# Autodesk Inventor assembly: OpticsTable_Shelf
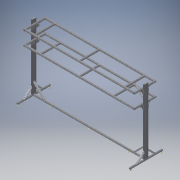
[picture p0: Inventor's stored thumbnail of the model, 180x180]
Saved by Autodesk Inventor 2018 (Build 220112000, 112)
## iProperties
Created: 2018-01-27
Part Number: OpticsTable_Shelf
Document SubType Name: Assembly
Designer: Rich
Author: Rich
## Documents named in this file (23)
- C:\Users\Rich\development\UWaterloo\opticstable_shelf\OpticsTable_Shelf.iam
- C:\Users\Rich\development\UWaterloo\opticstable_shelf\8020-1545-S-1545-S X 54.ipt
- C:\Users\Rich\development\UWaterloo\opticstable_shelf\8020-1515-LS-1515-LS X 24.ipt
- C:\Users\Rich\development\UWaterloo\opticstable_shelf\8020-1515-LS-1515-LS X 21.ipt
- C:\Users\Rich\development\UWaterloo\opticstable_shelf\8020 Original Parts\8020-3660-DEFAULT.ipt
- C:\Users\Rich\development\UWaterloo\opticstable_shelf\8020-1515-LS-1515-LS X 36.ipt
- C:\Users\Rich\development\UWaterloo\opticstable_shelf\8020 Original Parts\8020-2561-$PARTNUMBER.ipt
- C:\Users\Rich\development\UWaterloo\opticstable_shelf\8020 Original Parts\8020-2563-$PARTNUMBER.ipt
- C:\Users\Rich\development\UWaterloo\opticstable_shelf\8020 Original Parts\8020-2190-DEFAULT.ipt
- C:\Users\Rich\development\UWaterloo\opticstable_shelf\8020 Original Parts\8020-2200-DEFAULT.ipt
- C:\Users\Rich\development\UWaterloo\opticstable_shelf\8020 Original Parts\RS2000-410-12.ipt
- C:\Users\Rich\development\UWaterloo\opticstable_shelf\8020 Original Parts\Newport SL 1200-422.ipt
- C:\Users\Rich\development\UWaterloo\opticstable_shelf\8020-1515-LS-1515-LS X 120.ipt
- C:\Users\Rich\development\UWaterloo\opticstable_shelf\8020-1515-LS-1515-LS X 123.ipt
- C:\Users\Rich\development\UWaterloo\opticstable_shelf\8020 Original Parts\8020-3118-DEFAULT.ipt
- C:\Users\Rich\development\UWaterloo\opticstable_shelf\8020 Original Parts\8020-4461-DEFAULT.ipt
- C:\Users\Rich\development\UWaterloo\opticstable_shelf\8020 Original Parts\8020-4336-BLACK-DEFAULT.ipt
- C:\Users\Rich\development\UWaterloo\opticstable_shelf\8020 Original Parts\User Library-ANSI - BHCS - 0.625_5.5.ipt
- C:\Users\Rich\development\UWaterloo\opticstable_shelf\8020 Original Parts\8020-3202-DEFAULT.ipt
- C:\Users\Rich\development\UWaterloo\opticstable_shelf\8020 Original Parts\8020-3065-DEFAULT.ipt
- C:\Users\Rich\development\UWaterloo\opticstable_shelf\8020 Original Parts\8020-2046-DEFAULT.ipt
- C:\Users\Rich\development\UWaterloo\opticstable_shelf\8020 Original Parts\8020-2030-Plain-DEFAULT.ipt
- C:\Users\Rich\development\UWaterloo\opticstable_shelf\8020 Original Parts\8020-3214-DEFAULT.ipt
## Components (176 placed, 22 different names)
1. 8020-1545-S-1545-S X 54:1 — Mate:12, Flush:22, Flush:26, Mate:18, Mate:25, Flush:29, Mate:26, Flush:33, Flush:41, Mate:36, Angle:10, Flush:42, Mate:37, Angle:11, Mate:50, Flush:53, Mate:81, Mate:82, Mate:118, Mate:120, Mate:167, Mate:168, Mate:169, Mate:337, Mate:338, Mate:339, Mate:340
2. 8020-1545-S-1545-S X 54:2 — Mate:205, Flush:97, Mate:206, Mate:207, Mate:208, Flush:98, Mate:209, Mate:210, Mate:211, Tangent:5, Mate:212, Mate:213, Mate:285, Mate:286, Mate:287, Mate:288, Mate:341, Flush:126, Flush:127
3. 8020-1515-LS-1515-LS X 36:1 — Mate:12, Flush:19, Flush:22, Mate:24, Mate:27, Flush:30, Mate:38, Flush:43, Mate:39, Flush:44, Flush:77, Mate:75, Mate:175, Flush:85, Flush:86, Mate:176, Flush:87, Flush:88
4. 8020-1515-LS-1515-LS X 36:2 — Mate:1, Flush:19, Mate:20, Mate:22, Flush:28, Mate:40, Flush:45, Mate:41, Flush:46, Mate:72, Flush:75, Mate:173, Flush:81, Flush:82, Mate:174, Flush:83, Flush:84, Mate:205, Flush:97, Flush:98
5. 8020-2561-$PARTNUMBER:1 — Mate:22, Flush:28
6. 8020-2561-$PARTNUMBER:2 — Mate:24, Mate:25, Flush:29
7. 8020-2563-$PARTNUMBER:1 — Mate:17, Tangent:1, Mate:67, Mate:211, Tangent:5
8. 8020-2563-$PARTNUMBER:2 — Mate:18, Mate:19, Flush:33, Mate:68, Tangent:2
9. 8020-2561-$PARTNUMBER:3 — Mate:26, Mate:27, Flush:30
10. 8020-2561-$PARTNUMBER:4 — Mate:20
11. 8020-2190-DEFAULT:1
12. 8020-2190-DEFAULT:2
13. 8020-2190-DEFAULT:3
14. 8020-3660-DEFAULT:9
15. 8020-3660-DEFAULT:10
16. 8020-3660-DEFAULT:11 — Flush:41, Mate:36, Angle:10
17. 8020-3660-DEFAULT:12 — Flush:42, Mate:37, Angle:11
18. 8020-2200-DEFAULT:1 — Mate:38, Flush:43
19. 8020-2200-DEFAULT:2 — Mate:39, Flush:44
20. 8020-2200-DEFAULT:3 — Mate:40, Flush:45
21. 8020-2200-DEFAULT:4 — Mate:41, Flush:46
22. 8020-2563-$PARTNUMBER:3 — Flush:76, Mate:73
23. 8020-2563-$PARTNUMBER:4 — Mate:50, Flush:53, Mate:74
24. 8020-2200-DEFAULT:5 — Mate:76, Flush:78
25. 8020-2200-DEFAULT:6 — Flush:79, Mate:77
26. RS2000-410-12:1 — Mate:57, Mate:58, Flush:60
27. 8020-1515-LS-1515-LS X 123:1 — Mate:72, Flush:75, Flush:76, Mate:73, Mate:74, Flush:77, Mate:75, Mate:76, Flush:78, Flush:79, Mate:77, Mate:78, Flush:80
28. 8020-2200-DEFAULT:7 — Mate:78, Flush:80
29. 8020-2046-DEFAULT:1 — Mate:167, Mate:168, Mate:169
30. 8020-2046-DEFAULT:2 — Mate:206, Mate:207, Mate:208
31. 8020-2030-Plain-DEFAULT:5 — Mate:173, Flush:81, Flush:82
32. 8020-2030-Plain-DEFAULT:6 — Mate:174, Flush:83, Flush:84
33. 8020-2030-Plain-DEFAULT:7 — Mate:175, Flush:85, Flush:86
34. 8020-2030-Plain-DEFAULT:8 — Mate:176, Flush:87, Flush:88
35. 8020-1515-LS-1515-LS X 24:1 — Flush:61, Mate:60, Flush:62, Mate:61, Flush:63, Flush:64, Mate:129, Mate:179, Flush:93, Flush:94, Mate:180, Flush:95, Flush:96
36. 8020-1515-LS-1515-LS X 24:2 — Flush:23, Flush:68, Mate:64, Flush:69, Mate:130, Mate:177, Flush:89, Flush:90, Flush:91, Mate:178, Flush:92, Flush:127
37. 8020-1515-LS-1515-LS X 21:1 — Mate:17, Mate:46, Flush:51, Angle:16, Mate:47, Mate:48, Angle:17, Flush:72, Mate:68, Tangent:2, Mate:71
38. 8020-1515-LS-1515-LS X 21:2 — Flush:23, Mate:44, Flush:49, Angle:14, Mate:45, Flush:50, Angle:15, Flush:67, Mate:63
39. 8020-1515-LS-1515-LS X 21:3 — Mate:19, Flush:47, Mate:42, Angle:12, Flush:48, Mate:43, Angle:13, Mate:62, Flush:65, Tangent:1, Mate:67
40. 8020-3660-DEFAULT:1 — Mate:66, Flush:71, Angle:18
41. 8020-3660-DEFAULT:2 — Mate:69, Flush:73, Angle:19
42. 8020-3660-DEFAULT:3 — Mate:70, Flush:74, Angle:20
43. 8020-3660-DEFAULT:4 — Mate:65, Flush:70
44. 8020-3660-DEFAULT:13 — Flush:47, Mate:42, Angle:12
45. 8020-3660-DEFAULT:14 — Flush:48, Mate:43, Angle:13
46. 8020-3660-DEFAULT:15 — Mate:44, Flush:49, Angle:14
47. 8020-3660-DEFAULT:16 — Mate:45, Flush:50, Angle:15
48. 8020-3660-DEFAULT:17 — Mate:46, Flush:51, Angle:16
49. 8020-3660-DEFAULT:18 — Mate:47, Mate:48, Angle:17
50. 8020-1515-LS-1515-LS X 120:1 — Flush:62, Mate:61, Flush:63, Mate:63, Mate:66, Flush:71, Angle:18, Mate:69, Flush:73, Angle:19, Mate:71
51. 8020-1515-LS-1515-LS X 120:2 — Flush:61, Mate:60, Flush:64, Mate:62, Flush:65, Flush:67, Flush:68, Mate:64, Flush:69, Mate:65, Flush:70, Flush:72, Mate:70, Flush:74, Angle:20
52. 8020-2030-Plain-DEFAULT:1 — Mate:180, Flush:95, Flush:96
53. 8020-2030-Plain-DEFAULT:2 — Mate:179, Flush:93, Flush:94
54. 8020-2030-Plain-DEFAULT:3 — Flush:91, Mate:178, Flush:92
55. 8020-2030-Plain-DEFAULT:4 — Mate:177, Flush:89, Flush:90
56. 8020-3118-DEFAULT:1 — Mate:84, Mate:85, Mate:88, Mate:184
57. 8020-4461-DEFAULT:1 — Mate:95, Mate:96, Mate:97, Mate:116, Mate:117, Mate:123, Mate:124, Mate:193, Mate:194, Mate:213
58. 8020-4461-DEFAULT:2 — Mate:83, Mate:88, Mate:89, Mate:127, Mate:128, Mate:195, Mate:196, Mate:198, Mate:200, Mate:212
59. 8020-4336-BLACK-DEFAULT:1 — Mate:83, Mate:84, Mate:85, Mate:86, Mate:87, Mate:130, Mate:149, Mate:150, Mate:154, Mate:155, Mate:156
60. 8020-3118-DEFAULT:2 — Mate:86, Mate:87, Mate:89, Mate:185
61. 8020-4336-BLACK-DEFAULT:2 — Mate:91, Mate:92, Mate:93, Mate:94, Mate:95, Mate:151, Mate:152, Mate:153, Mate:157, Mate:158
62. 8020-3118-DEFAULT:3 — Mate:91, Mate:92, Mate:97, Mate:186
63. 8020-3118-DEFAULT:4 — Mate:93, Mate:94, Mate:96, Mate:187
64. User Library-ANSI - BHCS - 0.625_5.5:3 — Mate:117, Mate:124, Mate:128, Mate:199, Mate:210
65. User Library-ANSI - BHCS - 0.625_5.5:4 — Mate:116, Mate:123, Mate:127, Mate:197, Mate:209
66. 8020-3202-DEFAULT:6
67. 8020-3065-DEFAULT:6 — Mate:151, Mate:157, Mate:158
68. 8020-3202-DEFAULT:7
69. 8020-3065-DEFAULT:7 — Mate:150, Mate:155, Mate:156
70. 8020-3202-DEFAULT:8
71. 8020-3065-DEFAULT:8 — Mate:149, Mate:154
72. 8020-3202-DEFAULT:9
73. 8020-3065-DEFAULT:9 — Mate:152, Mate:153
74. 8020-3214-DEFAULT:4 — Mate:185, Mate:196
75. 8020-3214-DEFAULT:5 — Mate:184, Mate:195
76. 8020-3214-DEFAULT:6 — Mate:186, Mate:193
77. 8020-3214-DEFAULT:7 — Mate:187, Mate:194
78. 8020-3214-DEFAULT:9 — Mate:197, Mate:198
79. 8020-3214-DEFAULT:10 — Mate:199, Mate:200
80. 8020-4461-DEFAULT:3 — Mate:81, Mate:109, Mate:110, Mate:111, Mate:112, Mate:114, Mate:115, Mate:119, Mate:189, Mate:190
81. 8020-4461-DEFAULT:4 — Mate:82, Mate:102, Mate:103, Mate:104, Mate:121, Mate:122, Mate:191, Mate:192, Mate:202, Mate:204
82. 8020-3118-DEFAULT:5 — Mate:98, Mate:99, Mate:104, Mate:181
83. 8020-4336-BLACK-DEFAULT:3 — Mate:98, Mate:99, Mate:100, Mate:101, Mate:102, Mate:129, Mate:159, Mate:160, Mate:161, Mate:162
84. 8020-3118-DEFAULT:6 — Mate:100, Mate:101, Mate:103, Mate:182
85. 8020-4336-BLACK-DEFAULT:4 — Mate:105, Mate:106, Mate:107, Mate:108, Mate:109, Mate:163, Mate:164, Mate:165, Mate:166
86. 8020-3118-DEFAULT:7 — Mate:105, Mate:106, Mate:110, Mate:183
87. 8020-3118-DEFAULT:8 — Mate:107, Mate:108, Mate:111, Mate:188
88. User Library-ANSI - BHCS - 0.625_5.5:1 — Mate:114, Mate:115, Mate:118, Mate:121, Mate:203
89. User Library-ANSI - BHCS - 0.625_5.5:2 — Mate:112, Mate:119, Mate:120, Mate:122, Mate:201
90. 8020-3202-DEFAULT:1 — Mate:131, Mate:132
91. 8020-3065-DEFAULT:1 — Mate:131, Mate:132, Mate:159, Mate:160
92. 8020-3202-DEFAULT:2
93. 8020-3065-DEFAULT:2 — Mate:163, Mate:164
94. 8020-3202-DEFAULT:4
95. 8020-3065-DEFAULT:4 — Mate:165, Mate:166
96. 8020-3202-DEFAULT:5
97. 8020-3065-DEFAULT:5 — Mate:161, Mate:162
98. 8020-3214-DEFAULT:1 — Mate:181, Mate:191
99. 8020-3214-DEFAULT:2 — Mate:182, Mate:192
100. 8020-3214-DEFAULT:3 — Mate:183, Mate:190
101. 8020-3214-DEFAULT:8 — Mate:188, Mate:189
102. 8020-3214-DEFAULT:11 — Mate:201, Mate:202
103. 8020-3214-DEFAULT:12 — Mate:203, Mate:204
104. 8020-1515-LS-1515-LS X 24:3
105. 8020-1515-LS-1515-LS X 24:4 — Mate:341, Mate:342, Flush:126
106. 8020-1515-LS-1515-LS X 21:4
107. 8020-1515-LS-1515-LS X 21:5
108. 8020-1515-LS-1515-LS X 21:6
109. 8020-3660-DEFAULT:19
110. 8020-3660-DEFAULT:20
111. 8020-3660-DEFAULT:21
112. 8020-3660-DEFAULT:22
113. 8020-3660-DEFAULT:23
114. 8020-3660-DEFAULT:24
115. 8020-3660-DEFAULT:25
116. 8020-3660-DEFAULT:26
117. 8020-3660-DEFAULT:27
118. 8020-3660-DEFAULT:28
119. 8020-1515-LS-1515-LS X 120:3
120. 8020-1515-LS-1515-LS X 120:4
121. 8020-2030-Plain-DEFAULT:9
122. 8020-2030-Plain-DEFAULT:10
123. 8020-2030-Plain-DEFAULT:11
124. 8020-2030-Plain-DEFAULT:12
125. 8020-3118-DEFAULT:9
126. 8020-4461-DEFAULT:5 — Mate:286
127. 8020-4461-DEFAULT:6 — Mate:285
128. 8020-4336-BLACK-DEFAULT:5
129. 8020-3118-DEFAULT:10
130. 8020-4336-BLACK-DEFAULT:6 — Mate:342
131. 8020-3118-DEFAULT:11
132. 8020-3118-DEFAULT:12
133. User Library-ANSI - BHCS - 0.625_5.5:5 — Mate:287
134. User Library-ANSI - BHCS - 0.625_5.5:6 — Mate:288
135. 8020-3202-DEFAULT:10
136. 8020-3065-DEFAULT:10
137. 8020-3202-DEFAULT:11
138. 8020-3065-DEFAULT:11
139. 8020-3202-DEFAULT:12
140. 8020-3065-DEFAULT:12
141. 8020-3202-DEFAULT:13
142. 8020-3065-DEFAULT:13
143. 8020-3214-DEFAULT:13
144. 8020-3214-DEFAULT:14
145. 8020-3214-DEFAULT:15
146. 8020-3214-DEFAULT:16
147. 8020-3214-DEFAULT:17
148. 8020-3214-DEFAULT:18
149. 8020-4461-DEFAULT:7 — Mate:338
150. 8020-4461-DEFAULT:8 — Mate:337
151. 8020-3118-DEFAULT:13
152. 8020-4336-BLACK-DEFAULT:7
153. 8020-3118-DEFAULT:14
154. 8020-4336-BLACK-DEFAULT:8
155. 8020-3118-DEFAULT:15
156. 8020-3118-DEFAULT:16
157. User Library-ANSI - BHCS - 0.625_5.5:7 — Mate:339
158. User Library-ANSI - BHCS - 0.625_5.5:8 — Mate:340
159. 8020-3202-DEFAULT:14
160. 8020-3065-DEFAULT:14
161. 8020-3202-DEFAULT:15
162. 8020-3065-DEFAULT:15
163. 8020-3202-DEFAULT:16
164. 8020-3065-DEFAULT:16
165. 8020-3202-DEFAULT:17
166. 8020-3065-DEFAULT:17
167. 8020-3214-DEFAULT:19
168. 8020-3214-DEFAULT:20
169. 8020-3214-DEFAULT:21
170. 8020-3214-DEFAULT:22
171. 8020-3214-DEFAULT:23
172. 8020-3214-DEFAULT:24
173. Newport SL 1200-422:1 — Mate:57, Mate:58, Flush:60, Mate:59
174. Newport SL 1200-422:2
175. Newport SL 1200-422:3
176. Newport SL 1200-422:4
## Component patterns: (4 elements, first: Newport SL 1200-422:1)
## Relationships (410: Mate 300, Flush 87, Angle 20, Tangent 3)
- Mate:1: 8020-1515-LS-1515-LS X 36:2
- Mate:12: 8020-1545-S-1545-S X 54:1 ↔ 8020-1515-LS-1515-LS X 36:1
- Flush:19: 8020-1515-LS-1515-LS X 36:1 ↔ 8020-1515-LS-1515-LS X 36:2
- Flush:22: 8020-1545-S-1545-S X 54:1 ↔ 8020-1515-LS-1515-LS X 36:1
- Flush:23 (-1530.95 mm): 8020-1515-LS-1515-LS X 24:2 ↔ 8020-1515-LS-1515-LS X 21:2
- Flush:26: 8020-1545-S-1545-S X 54:1
- Mate:17: 8020-2563-$PARTNUMBER:1 ↔ 8020-1515-LS-1515-LS X 21:1
- Mate:18: 8020-1545-S-1545-S X 54:1 ↔ 8020-2563-$PARTNUMBER:2
- Mate:19: 8020-2563-$PARTNUMBER:2 ↔ 8020-1515-LS-1515-LS X 21:3
- Mate:20: 8020-1515-LS-1515-LS X 36:2 ↔ 8020-2561-$PARTNUMBER:4
- Mate:22: 8020-1515-LS-1515-LS X 36:2 ↔ 8020-2561-$PARTNUMBER:1
- Flush:28: 8020-1515-LS-1515-LS X 36:2 ↔ 8020-2561-$PARTNUMBER:1
- Mate:24: 8020-1515-LS-1515-LS X 36:1 ↔ 8020-2561-$PARTNUMBER:2
- Mate:25: 8020-1545-S-1545-S X 54:1 ↔ 8020-2561-$PARTNUMBER:2
- Flush:29: 8020-1545-S-1545-S X 54:1 ↔ 8020-2561-$PARTNUMBER:2
- Mate:26: 8020-1545-S-1545-S X 54:1 ↔ 8020-2561-$PARTNUMBER:3
- Mate:27: 8020-1515-LS-1515-LS X 36:1 ↔ 8020-2561-$PARTNUMBER:3
- Flush:30: 8020-1515-LS-1515-LS X 36:1 ↔ 8020-2561-$PARTNUMBER:3
- Flush:33 (38.1 mm): 8020-1545-S-1545-S X 54:1 ↔ 8020-2563-$PARTNUMBER:2
- Flush:41: 8020-1545-S-1545-S X 54:1 ↔ 8020-3660-DEFAULT:11
- Mate:36: 8020-1545-S-1545-S X 54:1 ↔ 8020-3660-DEFAULT:11
- Angle:10 (180 deg): 8020-1545-S-1545-S X 54:1 ↔ 8020-3660-DEFAULT:11
- Flush:42: 8020-1545-S-1545-S X 54:1 ↔ 8020-3660-DEFAULT:12
- Mate:37: 8020-1545-S-1545-S X 54:1 ↔ 8020-3660-DEFAULT:12
- Angle:11 (180 deg): 8020-1545-S-1545-S X 54:1 ↔ 8020-3660-DEFAULT:12
- Mate:38: 8020-1515-LS-1515-LS X 36:1 ↔ 8020-2200-DEFAULT:1
- Flush:43 (-38.1 mm): 8020-1515-LS-1515-LS X 36:1 ↔ 8020-2200-DEFAULT:1
- Mate:39: 8020-1515-LS-1515-LS X 36:1 ↔ 8020-2200-DEFAULT:2
- Flush:44 (38.1 mm): 8020-1515-LS-1515-LS X 36:1 ↔ 8020-2200-DEFAULT:2
- Mate:40: 8020-1515-LS-1515-LS X 36:2 ↔ 8020-2200-DEFAULT:3
- Flush:45 (38.1 mm): 8020-1515-LS-1515-LS X 36:2 ↔ 8020-2200-DEFAULT:3
- Mate:41: 8020-1515-LS-1515-LS X 36:2 ↔ 8020-2200-DEFAULT:4
- Flush:46 (38.1 mm): 8020-1515-LS-1515-LS X 36:2 ↔ 8020-2200-DEFAULT:4
- Flush:47: 8020-1515-LS-1515-LS X 21:3 ↔ 8020-3660-DEFAULT:13
- Mate:42: 8020-1515-LS-1515-LS X 21:3 ↔ 8020-3660-DEFAULT:13
- Angle:12 (0 deg): 8020-1515-LS-1515-LS X 21:3 ↔ 8020-3660-DEFAULT:13
- Flush:48: 8020-1515-LS-1515-LS X 21:3 ↔ 8020-3660-DEFAULT:14
- Mate:43: 8020-1515-LS-1515-LS X 21:3 ↔ 8020-3660-DEFAULT:14
- Angle:13 (180 deg): 8020-1515-LS-1515-LS X 21:3 ↔ 8020-3660-DEFAULT:14
- Mate:44: 8020-1515-LS-1515-LS X 21:2 ↔ 8020-3660-DEFAULT:15
- Flush:49: 8020-1515-LS-1515-LS X 21:2 ↔ 8020-3660-DEFAULT:15
- Angle:14 (0 deg): 8020-1515-LS-1515-LS X 21:2 ↔ 8020-3660-DEFAULT:15
- Mate:45: 8020-1515-LS-1515-LS X 21:2 ↔ 8020-3660-DEFAULT:16
- Flush:50: 8020-1515-LS-1515-LS X 21:2 ↔ 8020-3660-DEFAULT:16
- Angle:15 (180 deg): 8020-1515-LS-1515-LS X 21:2 ↔ 8020-3660-DEFAULT:16
- Mate:46: 8020-1515-LS-1515-LS X 21:1 ↔ 8020-3660-DEFAULT:17
- Flush:51: 8020-1515-LS-1515-LS X 21:1 ↔ 8020-3660-DEFAULT:17
- Angle:16 (0 deg): 8020-1515-LS-1515-LS X 21:1 ↔ 8020-3660-DEFAULT:17
- Mate:47: 8020-1515-LS-1515-LS X 21:1 ↔ 8020-3660-DEFAULT:18
- Mate:48: 8020-1515-LS-1515-LS X 21:1 ↔ 8020-3660-DEFAULT:18
- Angle:17 (180 deg): 8020-1515-LS-1515-LS X 21:1 ↔ 8020-3660-DEFAULT:18
- Mate:50: 8020-1545-S-1545-S X 54:1 ↔ 8020-2563-$PARTNUMBER:4
- Flush:53 (38.1 mm): 8020-1545-S-1545-S X 54:1 ↔ 8020-2563-$PARTNUMBER:4
- Mate:57: RS2000-410-12:1 ↔ Newport SL 1200-422:1
- Mate:58 (-457.2 mm): RS2000-410-12:1 ↔ Newport SL 1200-422:1
- Flush:60 (254 mm): RS2000-410-12:1 ↔ Newport SL 1200-422:1
- Mate:59: Newport SL 1200-422:1
- Flush:61: 8020-1515-LS-1515-LS X 24:1 ↔ 8020-1515-LS-1515-LS X 120:2
- Mate:60: 8020-1515-LS-1515-LS X 24:1 ↔ 8020-1515-LS-1515-LS X 120:2
- Flush:62: 8020-1515-LS-1515-LS X 24:1 ↔ 8020-1515-LS-1515-LS X 120:1
- Mate:61: 8020-1515-LS-1515-LS X 24:1 ↔ 8020-1515-LS-1515-LS X 120:1
- Flush:63: 8020-1515-LS-1515-LS X 24:1 ↔ 8020-1515-LS-1515-LS X 120:1
- Flush:64: 8020-1515-LS-1515-LS X 24:1 ↔ 8020-1515-LS-1515-LS X 120:2
- Mate:62: 8020-1515-LS-1515-LS X 21:3 ↔ 8020-1515-LS-1515-LS X 120:2
- Flush:65: 8020-1515-LS-1515-LS X 21:3 ↔ 8020-1515-LS-1515-LS X 120:2
- Flush:67: 8020-1515-LS-1515-LS X 21:2 ↔ 8020-1515-LS-1515-LS X 120:2
- Mate:63: 8020-1515-LS-1515-LS X 21:2 ↔ 8020-1515-LS-1515-LS X 120:1
- Flush:68: 8020-1515-LS-1515-LS X 24:2 ↔ 8020-1515-LS-1515-LS X 120:2
- Mate:64: 8020-1515-LS-1515-LS X 24:2 ↔ 8020-1515-LS-1515-LS X 120:2
- Flush:69: 8020-1515-LS-1515-LS X 24:2 ↔ 8020-1515-LS-1515-LS X 120:2
- Mate:65: 8020-3660-DEFAULT:4 ↔ 8020-1515-LS-1515-LS X 120:2
- Flush:70: 8020-3660-DEFAULT:4 ↔ 8020-1515-LS-1515-LS X 120:2
- Mate:66: 8020-3660-DEFAULT:1 ↔ 8020-1515-LS-1515-LS X 120:1
- Flush:71: 8020-3660-DEFAULT:1 ↔ 8020-1515-LS-1515-LS X 120:1
- Angle:18 (0 deg): 8020-3660-DEFAULT:1 ↔ 8020-1515-LS-1515-LS X 120:1
- Tangent:1: 8020-2563-$PARTNUMBER:1 ↔ 8020-1515-LS-1515-LS X 21:3
- Mate:67: 8020-2563-$PARTNUMBER:1 ↔ 8020-1515-LS-1515-LS X 21:3
- Flush:72: 8020-1515-LS-1515-LS X 21:1 ↔ 8020-1515-LS-1515-LS X 120:2
- Mate:68: 8020-2563-$PARTNUMBER:2 ↔ 8020-1515-LS-1515-LS X 21:1
- Tangent:2: 8020-2563-$PARTNUMBER:2 ↔ 8020-1515-LS-1515-LS X 21:1
- Mate:69: 8020-3660-DEFAULT:2 ↔ 8020-1515-LS-1515-LS X 120:1
- Flush:73: 8020-3660-DEFAULT:2 ↔ 8020-1515-LS-1515-LS X 120:1
- Angle:19 (180 deg): 8020-3660-DEFAULT:2 ↔ 8020-1515-LS-1515-LS X 120:1
- Mate:70: 8020-3660-DEFAULT:3 ↔ 8020-1515-LS-1515-LS X 120:2
- Flush:74: 8020-3660-DEFAULT:3 ↔ 8020-1515-LS-1515-LS X 120:2
- Angle:20 (0 deg): 8020-3660-DEFAULT:3 ↔ 8020-1515-LS-1515-LS X 120:2
- Mate:71: 8020-1515-LS-1515-LS X 21:1 ↔ 8020-1515-LS-1515-LS X 120:1
- Mate:72: 8020-1515-LS-1515-LS X 36:2 ↔ 8020-1515-LS-1515-LS X 123:1
- Flush:75: 8020-1515-LS-1515-LS X 36:2 ↔ 8020-1515-LS-1515-LS X 123:1
- Flush:76: 8020-2563-$PARTNUMBER:3 ↔ 8020-1515-LS-1515-LS X 123:1
- Mate:73: 8020-2563-$PARTNUMBER:3 ↔ 8020-1515-LS-1515-LS X 123:1
- Mate:74: 8020-2563-$PARTNUMBER:4 ↔ 8020-1515-LS-1515-LS X 123:1
- Flush:77: 8020-1515-LS-1515-LS X 36:1 ↔ 8020-1515-LS-1515-LS X 123:1
- Mate:75: 8020-1515-LS-1515-LS X 36:1 ↔ 8020-1515-LS-1515-LS X 123:1
- Mate:76: 8020-2200-DEFAULT:5 ↔ 8020-1515-LS-1515-LS X 123:1
- Flush:78 (38.1 mm): 8020-2200-DEFAULT:5 ↔ 8020-1515-LS-1515-LS X 123:1
- Flush:79 (-38.1 mm): 8020-2200-DEFAULT:6 ↔ 8020-1515-LS-1515-LS X 123:1
- Mate:77: 8020-2200-DEFAULT:6 ↔ 8020-1515-LS-1515-LS X 123:1
- Mate:78: 8020-1515-LS-1515-LS X 123:1 ↔ 8020-2200-DEFAULT:7
- Flush:80 (38.1 mm): 8020-1515-LS-1515-LS X 123:1 ↔ 8020-2200-DEFAULT:7
- Mate:81: 8020-1545-S-1545-S X 54:1 ↔ 8020-4461-DEFAULT:3
- Mate:82: 8020-1545-S-1545-S X 54:1 ↔ 8020-4461-DEFAULT:4
- Mate:83: 8020-4461-DEFAULT:2 ↔ 8020-4336-BLACK-DEFAULT:1
- Mate:84: 8020-3118-DEFAULT:1 ↔ 8020-4336-BLACK-DEFAULT:1
- Mate:85: 8020-3118-DEFAULT:1 ↔ 8020-4336-BLACK-DEFAULT:1
- Mate:86: 8020-4336-BLACK-DEFAULT:1 ↔ 8020-3118-DEFAULT:2
- Mate:87: 8020-4336-BLACK-DEFAULT:1 ↔ 8020-3118-DEFAULT:2
- Mate:88: 8020-3118-DEFAULT:1 ↔ 8020-4461-DEFAULT:2
- Mate:89: 8020-4461-DEFAULT:2 ↔ 8020-3118-DEFAULT:2
- Mate:91: 8020-4336-BLACK-DEFAULT:2 ↔ 8020-3118-DEFAULT:3
- Mate:92: 8020-4336-BLACK-DEFAULT:2 ↔ 8020-3118-DEFAULT:3
- Mate:93: 8020-4336-BLACK-DEFAULT:2 ↔ 8020-3118-DEFAULT:4
- Mate:94: 8020-4336-BLACK-DEFAULT:2 ↔ 8020-3118-DEFAULT:4
- Mate:95: 8020-4461-DEFAULT:1 ↔ 8020-4336-BLACK-DEFAULT:2
- Mate:96: 8020-4461-DEFAULT:1 ↔ 8020-3118-DEFAULT:4
- Mate:97: 8020-4461-DEFAULT:1 ↔ 8020-3118-DEFAULT:3
- Mate:98: 8020-3118-DEFAULT:5 ↔ 8020-4336-BLACK-DEFAULT:3
- Mate:99: 8020-3118-DEFAULT:5 ↔ 8020-4336-BLACK-DEFAULT:3
- Mate:100: 8020-4336-BLACK-DEFAULT:3 ↔ 8020-3118-DEFAULT:6
- Mate:101: 8020-4336-BLACK-DEFAULT:3 ↔ 8020-3118-DEFAULT:6
- Mate:102: 8020-4461-DEFAULT:4 ↔ 8020-4336-BLACK-DEFAULT:3
- Mate:103: 8020-4461-DEFAULT:4 ↔ 8020-3118-DEFAULT:6
- Mate:104: 8020-4461-DEFAULT:4 ↔ 8020-3118-DEFAULT:5
- Mate:105: 8020-4336-BLACK-DEFAULT:4 ↔ 8020-3118-DEFAULT:7
- Mate:106: 8020-4336-BLACK-DEFAULT:4 ↔ 8020-3118-DEFAULT:7
- Mate:107: 8020-4336-BLACK-DEFAULT:4 ↔ 8020-3118-DEFAULT:8
- Mate:108: 8020-4336-BLACK-DEFAULT:4 ↔ 8020-3118-DEFAULT:8
- Mate:109: 8020-4461-DEFAULT:3 ↔ 8020-4336-BLACK-DEFAULT:4
- Mate:110: 8020-4461-DEFAULT:3 ↔ 8020-3118-DEFAULT:7
- Mate:111: 8020-4461-DEFAULT:3 ↔ 8020-3118-DEFAULT:8
- Mate:112: 8020-4461-DEFAULT:3 ↔ User Library-ANSI - BHCS - 0.625_5.5:2
- Mate:114: 8020-4461-DEFAULT:3 ↔ User Library-ANSI - BHCS - 0.625_5.5:1
- Mate:115: 8020-4461-DEFAULT:3 ↔ User Library-ANSI - BHCS - 0.625_5.5:1
- Mate:116: 8020-4461-DEFAULT:1 ↔ User Library-ANSI - BHCS - 0.625_5.5:4
- Mate:117: 8020-4461-DEFAULT:1 ↔ User Library-ANSI - BHCS - 0.625_5.5:3
- Mate:118: 8020-1545-S-1545-S X 54:1 ↔ User Library-ANSI - BHCS - 0.625_5.5:1
- Mate:119: 8020-4461-DEFAULT:3 ↔ User Library-ANSI - BHCS - 0.625_5.5:2
- Mate:120: 8020-1545-S-1545-S X 54:1 ↔ User Library-ANSI - BHCS - 0.625_5.5:2
- Mate:121: 8020-4461-DEFAULT:4 ↔ User Library-ANSI - BHCS - 0.625_5.5:1
- Mate:122: 8020-4461-DEFAULT:4 ↔ User Library-ANSI - BHCS - 0.625_5.5:2
- Mate:123: 8020-4461-DEFAULT:1 ↔ User Library-ANSI - BHCS - 0.625_5.5:4
- Mate:124: 8020-4461-DEFAULT:1 ↔ User Library-ANSI - BHCS - 0.625_5.5:3
- Mate:127: 8020-4461-DEFAULT:2 ↔ User Library-ANSI - BHCS - 0.625_5.5:4
- Mate:128: 8020-4461-DEFAULT:2 ↔ User Library-ANSI - BHCS - 0.625_5.5:3
- Mate:129: 8020-1515-LS-1515-LS X 24:1 ↔ 8020-4336-BLACK-DEFAULT:3
- Mate:130: 8020-1515-LS-1515-LS X 24:2 ↔ 8020-4336-BLACK-DEFAULT:1
- Mate:131: 8020-3202-DEFAULT:1 ↔ 8020-3065-DEFAULT:1
- Mate:132 (12.7 mm): 8020-3202-DEFAULT:1 ↔ 8020-3065-DEFAULT:1
- [Mate]: 8020-3202-DEFAULT:2 ↔ 8020-3065-DEFAULT:2
- [Mate] (12.7 mm): 8020-3202-DEFAULT:2 ↔ 8020-3065-DEFAULT:2
- [Mate]: 8020-3202-DEFAULT:4 ↔ 8020-3065-DEFAULT:4
- [Mate] (12.7 mm): 8020-3202-DEFAULT:4 ↔ 8020-3065-DEFAULT:4
- [Mate]: 8020-3202-DEFAULT:5 ↔ 8020-3065-DEFAULT:5
- [Mate] (12.7 mm): 8020-3202-DEFAULT:5 ↔ 8020-3065-DEFAULT:5
- [Mate]: 8020-3202-DEFAULT:6 ↔ 8020-3065-DEFAULT:6
- [Mate] (12.7 mm): 8020-3202-DEFAULT:6 ↔ 8020-3065-DEFAULT:6
- [Mate]: 8020-3202-DEFAULT:7 ↔ 8020-3065-DEFAULT:7
- [Mate] (12.7 mm): 8020-3202-DEFAULT:7 ↔ 8020-3065-DEFAULT:7
- [Mate]: 8020-3202-DEFAULT:8 ↔ 8020-3065-DEFAULT:8
- [Mate] (12.7 mm): 8020-3202-DEFAULT:8 ↔ 8020-3065-DEFAULT:8
- [Mate]: 8020-3202-DEFAULT:9 ↔ 8020-3065-DEFAULT:9
- [Mate] (12.7 mm): 8020-3202-DEFAULT:9 ↔ 8020-3065-DEFAULT:9
- Mate:149: 8020-4336-BLACK-DEFAULT:1 ↔ 8020-3065-DEFAULT:8
- Mate:150: 8020-4336-BLACK-DEFAULT:1 ↔ 8020-3065-DEFAULT:7
- Mate:151: 8020-4336-BLACK-DEFAULT:2 ↔ 8020-3065-DEFAULT:6
- Mate:152: 8020-4336-BLACK-DEFAULT:2 ↔ 8020-3065-DEFAULT:9
- Mate:153: 8020-4336-BLACK-DEFAULT:2 ↔ 8020-3065-DEFAULT:9
- Mate:154: 8020-4336-BLACK-DEFAULT:1 ↔ 8020-3065-DEFAULT:8
- Mate:155: 8020-4336-BLACK-DEFAULT:1 ↔ 8020-3065-DEFAULT:7
- Mate:156: 8020-4336-BLACK-DEFAULT:1 ↔ 8020-3065-DEFAULT:7
- Mate:157: 8020-4336-BLACK-DEFAULT:2 ↔ 8020-3065-DEFAULT:6
- Mate:158: 8020-4336-BLACK-DEFAULT:2 ↔ 8020-3065-DEFAULT:6
- Mate:159: 8020-4336-BLACK-DEFAULT:3 ↔ 8020-3065-DEFAULT:1
- Mate:160: 8020-4336-BLACK-DEFAULT:3 ↔ 8020-3065-DEFAULT:1
- Mate:161: 8020-4336-BLACK-DEFAULT:3 ↔ 8020-3065-DEFAULT:5
- Mate:162: 8020-4336-BLACK-DEFAULT:3 ↔ 8020-3065-DEFAULT:5
- Mate:163: 8020-4336-BLACK-DEFAULT:4 ↔ 8020-3065-DEFAULT:2
- Mate:164: 8020-4336-BLACK-DEFAULT:4 ↔ 8020-3065-DEFAULT:2
- Mate:165: 8020-4336-BLACK-DEFAULT:4 ↔ 8020-3065-DEFAULT:4
- Mate:166: 8020-4336-BLACK-DEFAULT:4 ↔ 8020-3065-DEFAULT:4
- Mate:167: 8020-1545-S-1545-S X 54:1 ↔ 8020-2046-DEFAULT:1
- Mate:168: 8020-1545-S-1545-S X 54:1 ↔ 8020-2046-DEFAULT:1
- Mate:169: 8020-1545-S-1545-S X 54:1 ↔ 8020-2046-DEFAULT:1
- Mate:173: 8020-1515-LS-1515-LS X 36:2 ↔ 8020-2030-Plain-DEFAULT:5
- Flush:81: 8020-1515-LS-1515-LS X 36:2 ↔ 8020-2030-Plain-DEFAULT:5
- Flush:82: 8020-1515-LS-1515-LS X 36:2 ↔ 8020-2030-Plain-DEFAULT:5
- Mate:174: 8020-1515-LS-1515-LS X 36:2 ↔ 8020-2030-Plain-DEFAULT:6
- Flush:83: 8020-1515-LS-1515-LS X 36:2 ↔ 8020-2030-Plain-DEFAULT:6
- Flush:84: 8020-1515-LS-1515-LS X 36:2 ↔ 8020-2030-Plain-DEFAULT:6
- Mate:175: 8020-1515-LS-1515-LS X 36:1 ↔ 8020-2030-Plain-DEFAULT:7
- Flush:85: 8020-1515-LS-1515-LS X 36:1 ↔ 8020-2030-Plain-DEFAULT:7
- Flush:86: 8020-1515-LS-1515-LS X 36:1 ↔ 8020-2030-Plain-DEFAULT:7
- Mate:176: 8020-1515-LS-1515-LS X 36:1 ↔ 8020-2030-Plain-DEFAULT:8
- Flush:87: 8020-1515-LS-1515-LS X 36:1 ↔ 8020-2030-Plain-DEFAULT:8
- Flush:88: 8020-1515-LS-1515-LS X 36:1 ↔ 8020-2030-Plain-DEFAULT:8
- Mate:177: 8020-1515-LS-1515-LS X 24:2 ↔ 8020-2030-Plain-DEFAULT:4
- Flush:89: 8020-1515-LS-1515-LS X 24:2 ↔ 8020-2030-Plain-DEFAULT:4
- Flush:90: 8020-1515-LS-1515-LS X 24:2 ↔ 8020-2030-Plain-DEFAULT:4
- Flush:91: 8020-1515-LS-1515-LS X 24:2 ↔ 8020-2030-Plain-DEFAULT:3
- Mate:178: 8020-1515-LS-1515-LS X 24:2 ↔ 8020-2030-Plain-DEFAULT:3
- Flush:92: 8020-1515-LS-1515-LS X 24:2 ↔ 8020-2030-Plain-DEFAULT:3
- Mate:179: 8020-1515-LS-1515-LS X 24:1 ↔ 8020-2030-Plain-DEFAULT:2
- Flush:93: 8020-1515-LS-1515-LS X 24:1 ↔ 8020-2030-Plain-DEFAULT:2
- Flush:94: 8020-1515-LS-1515-LS X 24:1 ↔ 8020-2030-Plain-DEFAULT:2
- Mate:180: 8020-1515-LS-1515-LS X 24:1 ↔ 8020-2030-Plain-DEFAULT:1
- Flush:95: 8020-1515-LS-1515-LS X 24:1 ↔ 8020-2030-Plain-DEFAULT:1
- Flush:96: 8020-1515-LS-1515-LS X 24:1 ↔ 8020-2030-Plain-DEFAULT:1
- Mate:181: 8020-3118-DEFAULT:5 ↔ 8020-3214-DEFAULT:1
- Mate:182: 8020-3118-DEFAULT:6 ↔ 8020-3214-DEFAULT:2
- Mate:183: 8020-3118-DEFAULT:7 ↔ 8020-3214-DEFAULT:3
- Mate:184: 8020-3118-DEFAULT:1 ↔ 8020-3214-DEFAULT:5
- Mate:185: 8020-3118-DEFAULT:2 ↔ 8020-3214-DEFAULT:4
- Mate:186: 8020-3118-DEFAULT:3 ↔ 8020-3214-DEFAULT:6
- Mate:187: 8020-3118-DEFAULT:4 ↔ 8020-3214-DEFAULT:7
- Mate:188: 8020-3118-DEFAULT:8 ↔ 8020-3214-DEFAULT:8
- Mate:189: 8020-4461-DEFAULT:3 ↔ 8020-3214-DEFAULT:8
- Mate:190: 8020-4461-DEFAULT:3 ↔ 8020-3214-DEFAULT:3
- Mate:191: 8020-4461-DEFAULT:4 ↔ 8020-3214-DEFAULT:1
- Mate:192: 8020-4461-DEFAULT:4 ↔ 8020-3214-DEFAULT:2
- Mate:193: 8020-4461-DEFAULT:1 ↔ 8020-3214-DEFAULT:6
- Mate:194: 8020-4461-DEFAULT:1 ↔ 8020-3214-DEFAULT:7
- Mate:195: 8020-4461-DEFAULT:2 ↔ 8020-3214-DEFAULT:5
- Mate:196: 8020-4461-DEFAULT:2 ↔ 8020-3214-DEFAULT:4
- Mate:197: User Library-ANSI - BHCS - 0.625_5.5:4 ↔ 8020-3214-DEFAULT:9
- Mate:198: 8020-4461-DEFAULT:2 ↔ 8020-3214-DEFAULT:9
- Mate:199: User Library-ANSI - BHCS - 0.625_5.5:3 ↔ 8020-3214-DEFAULT:10
- Mate:200: 8020-4461-DEFAULT:2 ↔ 8020-3214-DEFAULT:10
- Mate:201: User Library-ANSI - BHCS - 0.625_5.5:2 ↔ 8020-3214-DEFAULT:11
- Mate:202: 8020-4461-DEFAULT:4 ↔ 8020-3214-DEFAULT:11
- Mate:203: User Library-ANSI - BHCS - 0.625_5.5:1 ↔ 8020-3214-DEFAULT:12
- Mate:204: 8020-4461-DEFAULT:4 ↔ 8020-3214-DEFAULT:12
- Mate:205: 8020-1545-S-1545-S X 54:2 ↔ 8020-1515-LS-1515-LS X 36:2
- Flush:97: 8020-1545-S-1545-S X 54:2 ↔ 8020-1515-LS-1515-LS X 36:2
- Mate:206: 8020-1545-S-1545-S X 54:2 ↔ 8020-2046-DEFAULT:2
- Mate:207: 8020-1545-S-1545-S X 54:2 ↔ 8020-2046-DEFAULT:2
- Mate:208: 8020-1545-S-1545-S X 54:2 ↔ 8020-2046-DEFAULT:2
- Flush:98 (400.05 mm): 8020-1545-S-1545-S X 54:2 ↔ 8020-1515-LS-1515-LS X 36:2
- Mate:209: 8020-1545-S-1545-S X 54:2 ↔ User Library-ANSI - BHCS - 0.625_5.5:4
- Mate:210: 8020-1545-S-1545-S X 54:2 ↔ User Library-ANSI - BHCS - 0.625_5.5:3
- Mate:211: 8020-1545-S-1545-S X 54:2 ↔ 8020-2563-$PARTNUMBER:1
- Tangent:5: 8020-1545-S-1545-S X 54:2 ↔ 8020-2563-$PARTNUMBER:1
- Mate:212: 8020-1545-S-1545-S X 54:2 ↔ 8020-4461-DEFAULT:2
- Mate:213: 8020-1545-S-1545-S X 54:2 ↔ 8020-4461-DEFAULT:1
- [Flush] (-1530.95 mm): 8020-1515-LS-1515-LS X 24:4 ↔ 8020-1515-LS-1515-LS X 21:5
- [Flush]: 8020-1515-LS-1515-LS X 21:6 ↔ 8020-3660-DEFAULT:23
- [Mate]: 8020-1515-LS-1515-LS X 21:6 ↔ 8020-3660-DEFAULT:23
- [Angle] (0 deg): 8020-1515-LS-1515-LS X 21:6 ↔ 8020-3660-DEFAULT:23
- [Flush]: 8020-1515-LS-1515-LS X 21:6 ↔ 8020-3660-DEFAULT:24
- [Mate]: 8020-1515-LS-1515-LS X 21:6 ↔ 8020-3660-DEFAULT:24
- [Angle] (180 deg): 8020-1515-LS-1515-LS X 21:6 ↔ 8020-3660-DEFAULT:24
- [Mate]: 8020-1515-LS-1515-LS X 21:5 ↔ 8020-3660-DEFAULT:25
- [Flush]: 8020-1515-LS-1515-LS X 21:5 ↔ 8020-3660-DEFAULT:25
- [Angle] (0 deg): 8020-1515-LS-1515-LS X 21:5 ↔ 8020-3660-DEFAULT:25
- [Mate]: 8020-1515-LS-1515-LS X 21:5 ↔ 8020-3660-DEFAULT:26
- [Flush]: 8020-1515-LS-1515-LS X 21:5 ↔ 8020-3660-DEFAULT:26
- [Angle] (180 deg): 8020-1515-LS-1515-LS X 21:5 ↔ 8020-3660-DEFAULT:26
- [Mate]: 8020-1515-LS-1515-LS X 21:4 ↔ 8020-3660-DEFAULT:27
- [Flush]: 8020-1515-LS-1515-LS X 21:4 ↔ 8020-3660-DEFAULT:27
- [Angle] (0 deg): 8020-1515-LS-1515-LS X 21:4 ↔ 8020-3660-DEFAULT:27
- [Mate]: 8020-1515-LS-1515-LS X 21:4 ↔ 8020-3660-DEFAULT:28
- [Mate]: 8020-1515-LS-1515-LS X 21:4 ↔ 8020-3660-DEFAULT:28
- [Angle] (180 deg): 8020-1515-LS-1515-LS X 21:4 ↔ 8020-3660-DEFAULT:28
- [Flush]: 8020-1515-LS-1515-LS X 24:3 ↔ 8020-1515-LS-1515-LS X 120:4
- [Mate]: 8020-1515-LS-1515-LS X 24:3 ↔ 8020-1515-LS-1515-LS X 120:4
- [Flush]: 8020-1515-LS-1515-LS X 24:3 ↔ 8020-1515-LS-1515-LS X 120:3
- [Mate]: 8020-1515-LS-1515-LS X 24:3 ↔ 8020-1515-LS-1515-LS X 120:3
- [Flush]: 8020-1515-LS-1515-LS X 24:3 ↔ 8020-1515-LS-1515-LS X 120:3
- [Flush]: 8020-1515-LS-1515-LS X 24:3 ↔ 8020-1515-LS-1515-LS X 120:4
- [Mate]: 8020-1515-LS-1515-LS X 21:6 ↔ 8020-1515-LS-1515-LS X 120:4
- [Flush]: 8020-1515-LS-1515-LS X 21:6 ↔ 8020-1515-LS-1515-LS X 120:4
- [Flush]: 8020-1515-LS-1515-LS X 21:5 ↔ 8020-1515-LS-1515-LS X 120:4
- [Mate]: 8020-1515-LS-1515-LS X 21:5 ↔ 8020-1515-LS-1515-LS X 120:3
- [Flush]: 8020-1515-LS-1515-LS X 24:4 ↔ 8020-1515-LS-1515-LS X 120:4
- [Mate]: 8020-1515-LS-1515-LS X 24:4 ↔ 8020-1515-LS-1515-LS X 120:4
- [Flush]: 8020-1515-LS-1515-LS X 24:4 ↔ 8020-1515-LS-1515-LS X 120:4
- [Mate]: 8020-3660-DEFAULT:22 ↔ 8020-1515-LS-1515-LS X 120:4
- [Flush]: 8020-3660-DEFAULT:22 ↔ 8020-1515-LS-1515-LS X 120:4
- [Mate]: 8020-3660-DEFAULT:19 ↔ 8020-1515-LS-1515-LS X 120:3
- [Flush]: 8020-3660-DEFAULT:19 ↔ 8020-1515-LS-1515-LS X 120:3
- [Angle] (0 deg): 8020-3660-DEFAULT:19 ↔ 8020-1515-LS-1515-LS X 120:3
- [Flush]: 8020-1515-LS-1515-LS X 21:4 ↔ 8020-1515-LS-1515-LS X 120:4
- [Mate]: 8020-3660-DEFAULT:20 ↔ 8020-1515-LS-1515-LS X 120:3
- [Flush]: 8020-3660-DEFAULT:20 ↔ 8020-1515-LS-1515-LS X 120:3
- [Angle] (180 deg): 8020-3660-DEFAULT:20 ↔ 8020-1515-LS-1515-LS X 120:3
- [Mate]: 8020-3660-DEFAULT:21 ↔ 8020-1515-LS-1515-LS X 120:4
- [Flush]: 8020-3660-DEFAULT:21 ↔ 8020-1515-LS-1515-LS X 120:4
- [Angle] (0 deg): 8020-3660-DEFAULT:21 ↔ 8020-1515-LS-1515-LS X 120:4
- [Mate]: 8020-1515-LS-1515-LS X 21:4 ↔ 8020-1515-LS-1515-LS X 120:3
- [Mate]: 8020-1515-LS-1515-LS X 24:4 ↔ 8020-2030-Plain-DEFAULT:12
- [Flush]: 8020-1515-LS-1515-LS X 24:4 ↔ 8020-2030-Plain-DEFAULT:12
- [Flush]: 8020-1515-LS-1515-LS X 24:4 ↔ 8020-2030-Plain-DEFAULT:12
- [Flush]: 8020-1515-LS-1515-LS X 24:4 ↔ 8020-2030-Plain-DEFAULT:11
- [Mate]: 8020-1515-LS-1515-LS X 24:4 ↔ 8020-2030-Plain-DEFAULT:11
- [Flush]: 8020-1515-LS-1515-LS X 24:4 ↔ 8020-2030-Plain-DEFAULT:11
- [Mate]: 8020-1515-LS-1515-LS X 24:3 ↔ 8020-2030-Plain-DEFAULT:10
- [Flush]: 8020-1515-LS-1515-LS X 24:3 ↔ 8020-2030-Plain-DEFAULT:10
- [Flush]: 8020-1515-LS-1515-LS X 24:3 ↔ 8020-2030-Plain-DEFAULT:10
- [Mate]: 8020-1515-LS-1515-LS X 24:3 ↔ 8020-2030-Plain-DEFAULT:9
- [Flush]: 8020-1515-LS-1515-LS X 24:3 ↔ 8020-2030-Plain-DEFAULT:9
- [Flush]: 8020-1515-LS-1515-LS X 24:3 ↔ 8020-2030-Plain-DEFAULT:9
- [Mate]: 8020-4461-DEFAULT:6 ↔ 8020-4336-BLACK-DEFAULT:5
- [Mate]: 8020-3118-DEFAULT:9 ↔ 8020-4336-BLACK-DEFAULT:5
- [Mate]: 8020-3118-DEFAULT:9 ↔ 8020-4336-BLACK-DEFAULT:5
- [Mate]: 8020-4336-BLACK-DEFAULT:5 ↔ 8020-3118-DEFAULT:10
- [Mate]: 8020-4336-BLACK-DEFAULT:5 ↔ 8020-3118-DEFAULT:10
- [Mate]: 8020-3118-DEFAULT:9 ↔ 8020-4461-DEFAULT:6
- [Mate]: 8020-4461-DEFAULT:6 ↔ 8020-3118-DEFAULT:10
- [Mate]: 8020-4336-BLACK-DEFAULT:6 ↔ 8020-3118-DEFAULT:11
- [Mate]: 8020-4336-BLACK-DEFAULT:6 ↔ 8020-3118-DEFAULT:11
- [Mate]: 8020-4336-BLACK-DEFAULT:6 ↔ 8020-3118-DEFAULT:12
- [Mate]: 8020-4336-BLACK-DEFAULT:6 ↔ 8020-3118-DEFAULT:12
- [Mate]: 8020-4461-DEFAULT:5 ↔ 8020-4336-BLACK-DEFAULT:6
- [Mate]: 8020-4461-DEFAULT:5 ↔ 8020-3118-DEFAULT:12
- [Mate]: 8020-4461-DEFAULT:5 ↔ 8020-3118-DEFAULT:11
- [Mate]: 8020-4461-DEFAULT:5 ↔ User Library-ANSI - BHCS - 0.625_5.5:6
- [Mate]: 8020-4461-DEFAULT:5 ↔ User Library-ANSI - BHCS - 0.625_5.5:5
- [Mate]: 8020-4461-DEFAULT:5 ↔ User Library-ANSI - BHCS - 0.625_5.5:6
- [Mate]: 8020-4461-DEFAULT:5 ↔ User Library-ANSI - BHCS - 0.625_5.5:5
- [Mate]: 8020-4461-DEFAULT:6 ↔ User Library-ANSI - BHCS - 0.625_5.5:6
- [Mate]: 8020-4461-DEFAULT:6 ↔ User Library-ANSI - BHCS - 0.625_5.5:5
- [Mate]: 8020-3202-DEFAULT:10 ↔ 8020-3065-DEFAULT:10
- [Mate] (12.7 mm): 8020-3202-DEFAULT:10 ↔ 8020-3065-DEFAULT:10
- [Mate]: 8020-3202-DEFAULT:11 ↔ 8020-3065-DEFAULT:11
- [Mate] (12.7 mm): 8020-3202-DEFAULT:11 ↔ 8020-3065-DEFAULT:11
- [Mate]: 8020-3202-DEFAULT:12 ↔ 8020-3065-DEFAULT:12
- [Mate] (12.7 mm): 8020-3202-DEFAULT:12 ↔ 8020-3065-DEFAULT:12
- [Mate]: 8020-3202-DEFAULT:13 ↔ 8020-3065-DEFAULT:13
- [Mate] (12.7 mm): 8020-3202-DEFAULT:13 ↔ 8020-3065-DEFAULT:13
- [Mate]: 8020-4336-BLACK-DEFAULT:5 ↔ 8020-3065-DEFAULT:12
- [Mate]: 8020-4336-BLACK-DEFAULT:5 ↔ 8020-3065-DEFAULT:11
- [Mate]: 8020-4336-BLACK-DEFAULT:6 ↔ 8020-3065-DEFAULT:10
- [Mate]: 8020-4336-BLACK-DEFAULT:6 ↔ 8020-3065-DEFAULT:13
- [Mate]: 8020-4336-BLACK-DEFAULT:6 ↔ 8020-3065-DEFAULT:13
- [Mate]: 8020-4336-BLACK-DEFAULT:5 ↔ 8020-3065-DEFAULT:12
- [Mate]: 8020-4336-BLACK-DEFAULT:5 ↔ 8020-3065-DEFAULT:11
- [Mate]: 8020-4336-BLACK-DEFAULT:5 ↔ 8020-3065-DEFAULT:11
- [Mate]: 8020-4336-BLACK-DEFAULT:6 ↔ 8020-3065-DEFAULT:10
- [Mate]: 8020-4336-BLACK-DEFAULT:6 ↔ 8020-3065-DEFAULT:10
- [Mate]: 8020-3118-DEFAULT:9 ↔ 8020-3214-DEFAULT:14
- [Mate]: 8020-3118-DEFAULT:10 ↔ 8020-3214-DEFAULT:13
- [Mate]: 8020-3118-DEFAULT:11 ↔ 8020-3214-DEFAULT:15
- [Mate]: 8020-3118-DEFAULT:12 ↔ 8020-3214-DEFAULT:16
- [Mate]: 8020-4461-DEFAULT:5 ↔ 8020-3214-DEFAULT:15
- [Mate]: 8020-4461-DEFAULT:5 ↔ 8020-3214-DEFAULT:16
- [Mate]: 8020-4461-DEFAULT:6 ↔ 8020-3214-DEFAULT:14
- [Mate]: 8020-4461-DEFAULT:6 ↔ 8020-3214-DEFAULT:13
- [Mate]: User Library-ANSI - BHCS - 0.625_5.5:6 ↔ 8020-3214-DEFAULT:17
- [Mate]: 8020-4461-DEFAULT:6 ↔ 8020-3214-DEFAULT:17
- [Mate]: User Library-ANSI - BHCS - 0.625_5.5:5 ↔ 8020-3214-DEFAULT:18
- [Mate]: 8020-4461-DEFAULT:6 ↔ 8020-3214-DEFAULT:18
- Mate:285: 8020-1545-S-1545-S X 54:2 ↔ 8020-4461-DEFAULT:6
- Mate:286: 8020-1545-S-1545-S X 54:2 ↔ 8020-4461-DEFAULT:5
- Mate:287: 8020-1545-S-1545-S X 54:2 ↔ User Library-ANSI - BHCS - 0.625_5.5:5
- Mate:288: 8020-1545-S-1545-S X 54:2 ↔ User Library-ANSI - BHCS - 0.625_5.5:6
- [Mate]: 8020-3118-DEFAULT:13 ↔ 8020-4336-BLACK-DEFAULT:7
- [Mate]: 8020-3118-DEFAULT:13 ↔ 8020-4336-BLACK-DEFAULT:7
- [Mate]: 8020-4336-BLACK-DEFAULT:7 ↔ 8020-3118-DEFAULT:14
- [Mate]: 8020-4336-BLACK-DEFAULT:7 ↔ 8020-3118-DEFAULT:14
- [Mate]: 8020-4461-DEFAULT:8 ↔ 8020-4336-BLACK-DEFAULT:7
- [Mate]: 8020-4461-DEFAULT:8 ↔ 8020-3118-DEFAULT:14
- [Mate]: 8020-4461-DEFAULT:8 ↔ 8020-3118-DEFAULT:13
- [Mate]: 8020-4336-BLACK-DEFAULT:8 ↔ 8020-3118-DEFAULT:15
- [Mate]: 8020-4336-BLACK-DEFAULT:8 ↔ 8020-3118-DEFAULT:15
- [Mate]: 8020-4336-BLACK-DEFAULT:8 ↔ 8020-3118-DEFAULT:16
- [Mate]: 8020-4336-BLACK-DEFAULT:8 ↔ 8020-3118-DEFAULT:16
- [Mate]: 8020-4461-DEFAULT:7 ↔ 8020-4336-BLACK-DEFAULT:8
- [Mate]: 8020-4461-DEFAULT:7 ↔ 8020-3118-DEFAULT:15
- [Mate]: 8020-4461-DEFAULT:7 ↔ 8020-3118-DEFAULT:16
- [Mate]: 8020-4461-DEFAULT:7 ↔ User Library-ANSI - BHCS - 0.625_5.5:8
- [Mate]: 8020-4461-DEFAULT:7 ↔ User Library-ANSI - BHCS - 0.625_5.5:7
- [Mate]: 8020-4461-DEFAULT:7 ↔ User Library-ANSI - BHCS - 0.625_5.5:7
- [Mate]: 8020-4461-DEFAULT:7 ↔ User Library-ANSI - BHCS - 0.625_5.5:8
- [Mate]: 8020-4461-DEFAULT:8 ↔ User Library-ANSI - BHCS - 0.625_5.5:7
- [Mate]: 8020-4461-DEFAULT:8 ↔ User Library-ANSI - BHCS - 0.625_5.5:8
- [Mate]: 8020-3202-DEFAULT:14 ↔ 8020-3065-DEFAULT:14
- [Mate] (12.7 mm): 8020-3202-DEFAULT:14 ↔ 8020-3065-DEFAULT:14
- [Mate]: 8020-3202-DEFAULT:15 ↔ 8020-3065-DEFAULT:15
- [Mate] (12.7 mm): 8020-3202-DEFAULT:15 ↔ 8020-3065-DEFAULT:15
- [Mate]: 8020-3202-DEFAULT:16 ↔ 8020-3065-DEFAULT:16
- [Mate] (12.7 mm): 8020-3202-DEFAULT:16 ↔ 8020-3065-DEFAULT:16
- [Mate]: 8020-3202-DEFAULT:17 ↔ 8020-3065-DEFAULT:17
- [Mate] (12.7 mm): 8020-3202-DEFAULT:17 ↔ 8020-3065-DEFAULT:17
- [Mate]: 8020-4336-BLACK-DEFAULT:7 ↔ 8020-3065-DEFAULT:14
- [Mate]: 8020-4336-BLACK-DEFAULT:7 ↔ 8020-3065-DEFAULT:14
- [Mate]: 8020-4336-BLACK-DEFAULT:7 ↔ 8020-3065-DEFAULT:17
- [Mate]: 8020-4336-BLACK-DEFAULT:7 ↔ 8020-3065-DEFAULT:17
- [Mate]: 8020-4336-BLACK-DEFAULT:8 ↔ 8020-3065-DEFAULT:15
- [Mate]: 8020-4336-BLACK-DEFAULT:8 ↔ 8020-3065-DEFAULT:15
- [Mate]: 8020-4336-BLACK-DEFAULT:8 ↔ 8020-3065-DEFAULT:16
- [Mate]: 8020-4336-BLACK-DEFAULT:8 ↔ 8020-3065-DEFAULT:16
- [Mate]: 8020-3118-DEFAULT:13 ↔ 8020-3214-DEFAULT:19
- [Mate]: 8020-3118-DEFAULT:14 ↔ 8020-3214-DEFAULT:20
- [Mate]: 8020-3118-DEFAULT:15 ↔ 8020-3214-DEFAULT:21
- [Mate]: 8020-3118-DEFAULT:16 ↔ 8020-3214-DEFAULT:22
- [Mate]: 8020-4461-DEFAULT:7 ↔ 8020-3214-DEFAULT:22
- [Mate]: 8020-4461-DEFAULT:7 ↔ 8020-3214-DEFAULT:21
- [Mate]: 8020-4461-DEFAULT:8 ↔ 8020-3214-DEFAULT:19
- [Mate]: 8020-4461-DEFAULT:8 ↔ 8020-3214-DEFAULT:20
- [Mate]: User Library-ANSI - BHCS - 0.625_5.5:8 ↔ 8020-3214-DEFAULT:23
- [Mate]: 8020-4461-DEFAULT:8 ↔ 8020-3214-DEFAULT:23
- [Mate]: User Library-ANSI - BHCS - 0.625_5.5:7 ↔ 8020-3214-DEFAULT:24
- [Mate]: 8020-4461-DEFAULT:8 ↔ 8020-3214-DEFAULT:24
- Mate:337: 8020-1545-S-1545-S X 54:1 ↔ 8020-4461-DEFAULT:8
- Mate:338: 8020-1545-S-1545-S X 54:1 ↔ 8020-4461-DEFAULT:7
- Mate:339: 8020-1545-S-1545-S X 54:1 ↔ User Library-ANSI - BHCS - 0.625_5.5:7
- Mate:340: 8020-1545-S-1545-S X 54:1 ↔ User Library-ANSI - BHCS - 0.625_5.5:8
- Mate:341: 8020-1545-S-1545-S X 54:2 ↔ 8020-1515-LS-1515-LS X 24:4
- Mate:342: 8020-1515-LS-1515-LS X 24:4 ↔ 8020-4336-BLACK-DEFAULT:6
- Flush:126 (247.65 mm): 8020-1545-S-1545-S X 54:2 ↔ 8020-1515-LS-1515-LS X 24:4
- Flush:127 (247.65 mm): 8020-1545-S-1545-S X 54:2 ↔ 8020-1515-LS-1515-LS X 24:2
## Named parameters: d285_d283 = 0 mm, d286_d284 = 12.7 mm, d289_d285_d283 = 0 mm, d290_d286_d284 = 12.7 mm, d291_d285_d283 = 0 mm, d292_d286_d284 = 12.7 mm, d293_d285_d283 = 0 mm, d294_d286_d284 = 12.7 mm, d295_d285_d283 = 0 mm, d296_d286_d284 = 12.7 mm, d297_d285_d283 = 0 mm, d298_d286_d284 = 12.7 mm, d299_d285_d283 = 0 mm, d300_d286_d284 = 12.7 mm, d387_d342 = 0 mm, d388_d343 = 0 mm, d389_d344 = 0 mm, d390_d345 = 0 mm, d391_d346 = 0 mm, d392_d347 = 0 mm, d393_d348 = 0 mm, d394_d337 = 0 mm, d395_d338 = 0 mm, d396_d339 = 0 mm, d397_d340 = 0 mm, d398_d341 = 0 mm, d399_d170 = 0 mm, d400_d171 = 0 mm, d401_d172 = 0 mm, d402_d173 = 0 mm, d403_d174 = 0 mm, d404_d175 = 0 mm, d405_d176 = 0 mm, d406_d179 = 0 mm, d407_d180 = 0 mm, d408_d181 = 0 mm, d409_d182 = 0 mm, d410_d183 = 0 mm, d411_d184 = 0 mm, d412_d185 = 0 mm, d413_d186 = 0 mm, d414_d187 = 0 mm, d415_d188 = 0 deg, d416_d191 = 0 mm, d417_d194 = 0 mm, d418_d195 = 0 mm, d419_d196 = 180 deg, d420_d197 = 0 mm, d421_d198 = 0 mm, d422_d199 = 0 deg, d423_d200 = 0 mm, d424_d130 = 0 mm, d425_d131 = 0 mm, d426_d132 = 0 deg, d427_d133 = 0 mm, d428_d134 = 0 mm, d429_d135 = 180 deg, d430_d169 = 0 mm, d431_d118 = 0 mm, d432_d119 = 0 mm, d433_d120 = 0 deg, d434_d121 = 0 mm, d435_d122 = 0 mm, d436_d123 = 180 deg, d437_d124 = 0 mm, d438_d125 = 0 mm, d439_d126 = 0 deg, d440_d127 = 0 mm, d441_d128 = 0 mm, d442_d129 = 180 deg, d443_d51 = -1530.95 mm, d444_d353 = 0 mm, d445_d354 = 0 mm, d446_d355 = 0 mm, d447_d356 = 0 mm, d448_d362 = 0 mm, d449_d363 = 0 mm, d450_d364 = 0 mm, d451_d365 = 0 mm, d452_d366 = 0 mm, d453_d367 = 0 mm, d454_d368 = 0 mm, d455_d369 = 0 mm, d456_d277 = 0 mm, d457_d278 = 0 mm, d458_d293_d285_d283 = 0 mm, d459_d294_d286_d284 = 12.7 mm, d460_d295_d285_d283 = 0 mm, d461_d296_d286_d284 = 12.7 mm, d462_d297_d285_d283 = 0 mm, d463_d298_d286_d284 = 12.7 mm, d464_d299_d285_d283 = 0 mm, d465_d300_d286_d284 = 12.7 mm, d466_d301 = 0 mm, d467_d302 = 0 mm, d468_d303 = 0 mm, d469_d304 = 0 mm, d470_d305 = 0 mm, d471_d306 = 0 mm, d472_d307 = 0 mm, d473_d308 = 0 mm, d474_d309 = 0 mm, d475_d310 = 0 mm, d476_d234 = 0 mm, d477_d266 = 0 mm, d478_d267 = 0 mm, d479_d273 = 0 mm, d480_d274 = 0 mm, d481_d220 = 0 mm, d482_d221 = 0 mm, d483_d222 = 0 mm, d484_d223 = 0 mm, d485_d224 = 0 mm, d486_d225 = 0 mm, d487_d226 = 0 mm, d488_d228 = 0 mm, d489_d229 = 0 mm, d490_d230 = 0 mm, d491_d231 = 0 mm, d492_d232 = 0 mm, d493_d233 = 0 mm, d498_d370 = 0 mm, d499_d371 = 0 mm, d500_d372 = 0 mm, d501_d373 = 0 mm, d502_d350 = 0 mm, d503_d351 = 0 mm, d504_d352 = 0 mm, d505_d357 = 0 mm, d506_d358 = 0 mm, d507_d359 = 0 mm, d508_d360 = 0 mm, d509_d361 = 0 mm, d510_d314 = 0 mm, d511_d315 = 0 mm, d512_d316 = 0 mm, d513_d317 = 0 mm, d514_d318 = 0 mm, d515_d283 = 0 mm, d516_d284 = 12.7 mm, d517_d285_d283 = 0 mm, d518_d286_d284 = 12.7 mm, d519_d289_d285_d283 = 0 mm, d520_d290_d286_d284 = 12.7 mm, d521_d291_d285_d283 = 0 mm, d522_d292_d286_d284 = 12.7 mm, d523_d311 = 0 mm, d524_d312 = 0 mm, d525_d313 = 0 mm, d526_d235 = 0 mm, d527_d236 = 0 mm, d528_d237 = 0 mm, d529_d238 = 0 mm, d530_d239 = 0 mm, d531_d240 = 0 mm, d532_d241 = 0 mm, d533_d242 = 0 mm, d534_d243 = 0 mm, d535_d244 = 0 mm, d536_d245 = 0 mm, d537_d246 = 0 mm, d538_d247 = 0 mm, d539_d248 = 0 mm, d540_d262 = 0 mm, d541_d264 = 0 mm, d542_d265 = 0 mm, d543_d269 = 0 mm, d544_d271 = 0 mm, d545_d272 = 0 mm
